# Autodesk Inventor assembly: ASY Trommel
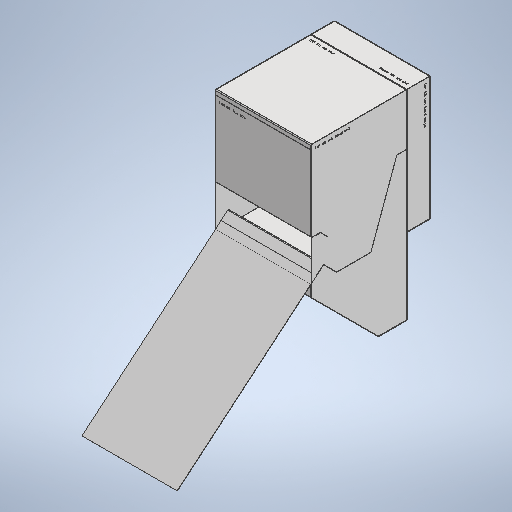
[picture p0: Inventor's stored thumbnail of the model, 512x512]
Saved by Autodesk Inventor 2025 (Build 290162010, 162A)
## iProperties
Created: 2024-08-07
Part Number: ASY Trommel
Document SubType Name: Assembly
Designer: pokla
Author: pokla
## Documents named in this file (16)
- C:\Users\pokla\Documents\Inventor\BSH_Beshkino_bio_tank\ASY Trommel.iam
- C:\Users\pokla\Documents\Inventor\BSH_Beshkino_bio_tank\TRM 011 bottom main.ipt
- C:\Users\pokla\Documents\Inventor\BSH_Beshkino_bio_tank\TRM 012 back main.ipt
- C:\Users\pokla\Documents\Inventor\BSH_Beshkino_bio_tank\TRM 013 top main.ipt
- C:\Users\pokla\Documents\Inventor\BSH_Beshkino_bio_tank\TRM 014 face main.ipt
- C:\Users\pokla\Documents\Inventor\BSH_Beshkino_bio_tank\TRM 015 left board main.ipt
- C:\Users\pokla\Documents\Inventor\BSH_Beshkino_bio_tank\TRM 016 right board main.ipt
- C:\Users\pokla\Documents\Inventor\BSH_Beshkino_bio_tank\TRM 017 sheet in.ipt
- C:\Users\pokla\Documents\Inventor\BSH_Beshkino_bio_tank\TRM 018 clipper.ipt
- C:\Users\pokla\Documents\Inventor\BSH_Beshkino_bio_tank\TRM 019 tray.ipt
- C:\Users\pokla\Documents\Inventor\BSH_Beshkino_bio_tank\021 TRM bottom damper.ipt
- C:\Users\pokla\Documents\Inventor\BSH_Beshkino_bio_tank\022 TRM back damper.ipt
- C:\Users\pokla\Documents\Inventor\BSH_Beshkino_bio_tank\023 TRM face damper.ipt
- C:\Users\pokla\Documents\Inventor\BSH_Beshkino_bio_tank\024 TRM top damper.ipt
- C:\Users\pokla\Documents\Inventor\BSH_Beshkino_bio_tank\025 TRM left board damper.ipt
- C:\Users\pokla\Documents\Inventor\BSH_Beshkino_bio_tank\026 TRM right board damper.ipt
## Components (15 placed, 15 different names)
1. TRM 011 bottom main:1 — Rigid:1
2. TRM 012 back main:1 — Rigid:1, Rigid:2, Mate:2, Rigid:13
3. TRM 013 top main:1 — Rigid:2, Rigid:3, Rigid:4, Rigid:5, Mate:1, Flush:1
4. TRM 014 face main:1 — Rigid:3, Rigid:6
5. TRM 015 left board main:1 — Rigid:4
6. TRM 016 right board main:1 — Rigid:5
7. TRM 017 sheet in:1 — Mate:1, Mate:2, Flush:1, Rigid:7
8. TRM 018 clipper:1 — Rigid:6
9. TRM 019 tray:1 — Rigid:7
10. 021 TRM bottom damper:1 — Rigid:8, Rigid:10, Rigid:11, Rigid:12
11. 022 TRM back damper:1 — Rigid:8, Rigid:9, Rigid:13
12. 023 TRM face damper:1 — Rigid:10
13. 024 TRM top damper:1 — Rigid:9
14. 025 TRM left board damper:1 — Rigid:11
15. 026 TRM right board damper:1 — Rigid:12
## Relationships (16: WeldJoint 13, Mate 2, Flush 1)
- Rigid:1 [WeldJoint]: TRM 011 bottom main:1 ↔ TRM 012 back main:1
- Rigid:2 [WeldJoint]: TRM 012 back main:1 ↔ TRM 013 top main:1
- Rigid:3 [WeldJoint]: TRM 013 top main:1 ↔ TRM 014 face main:1
- Rigid:4 [WeldJoint]: TRM 013 top main:1 ↔ TRM 015 left board main:1
- Rigid:5 [WeldJoint]: TRM 013 top main:1 ↔ TRM 016 right board main:1
- Mate:1 (270 mm): TRM 013 top main:1 ↔ TRM 017 sheet in:1
- Mate:2: TRM 012 back main:1 ↔ TRM 017 sheet in:1
- Flush:1: TRM 013 top main:1 ↔ TRM 017 sheet in:1
- Rigid:6 [WeldJoint]: TRM 014 face main:1 ↔ TRM 018 clipper:1
- Rigid:7 [WeldJoint]: TRM 017 sheet in:1 ↔ TRM 019 tray:1
- Rigid:8 [WeldJoint]: 021 TRM bottom damper:1 ↔ 022 TRM back damper:1
- Rigid:9 [WeldJoint]: 022 TRM back damper:1 ↔ 024 TRM top damper:1
- Rigid:10 [WeldJoint]: 021 TRM bottom damper:1 ↔ 023 TRM face damper:1
- Rigid:11 [WeldJoint]: 021 TRM bottom damper:1 ↔ 025 TRM left board damper:1
- Rigid:12 [WeldJoint]: 021 TRM bottom damper:1 ↔ 026 TRM right board damper:1
- Rigid:13 [WeldJoint]: TRM 012 back main:1 ↔ 022 TRM back damper:1
